# Autodesk Inventor assembly: E001_BancDeTest
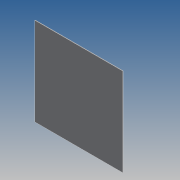
[picture p0: Inventor's stored thumbnail of the model, 180x180]
Saved by Autodesk Inventor 2020 (Build 240168000, 168)
## iProperties
Created: 2021-09-24
Part Number: E001_BancDeTest
Document SubType Name: Assembly
Designer: gabri
Author: gabri
## Documents named in this file (3)
- D:\PGA\E001_BancDeTest.iam
- D:\PGA\P002_plancher.ipt
- D:\PGA\P001_CageDeTest.ipt
## Components (2 placed, 2 different names)
1. P002_plancher:1 — Placage:1, Placage:2, Placage:3, Placage:4
2. P001_CageDeTest:1 — Placage:4
## Relationships (4: Mate 4)
- Placage:1 [Mate]: P002_plancher:1
- Placage:2 [Mate]: P002_plancher:1
- Placage:3 [Mate]: P002_plancher:1
- Placage:4 [Mate]: P002_plancher:1 ↔ P001_CageDeTest:1
